# Autodesk Inventor assembly: КВ33.044.900 - Клапан присоски впускной
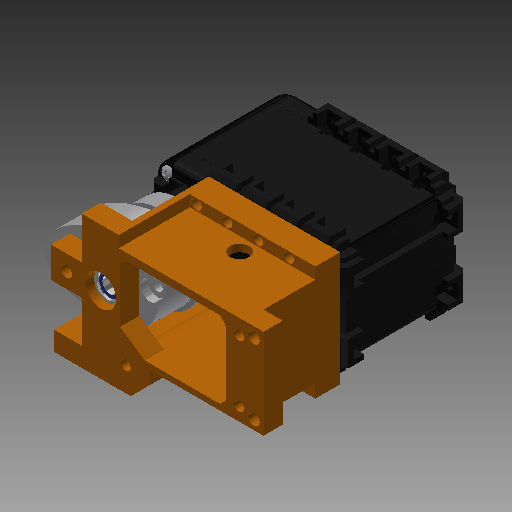
[picture p0: Inventor's stored thumbnail of the model, 512x512]
Saved by Autodesk Inventor 2019 (Build 230136000, 136)
## iProperties
Created: 2019-08-25
Part Number: КВ33.044.900 - Клапан присоски впускной
Material: Типовые
Document SubType Name: Assembly
Designer: Петров Иван
Mass: 93.2423 g
Surface Area: 263.543 cm^2
Volume: 60.5014 cm^3
Density: 1.54116 g/cm^3
Author: Петров Иван
## Documents named in this file (6)
- E:\IVAN\Kvantoriada2019\optimal_gripper\hardware\КВ33.044.900 - Клапан присоски впускной.iam
- E:\IVAN\Kvantoriada2019\optimal_gripper\hardware\КВ33.044.901  - Опора клапана присоски.ipt
- E:\IVAN\Kvantoriada2019\optimal_gripper\hardware\Стандартные изделия\Сервомотор Dynamixel AX-12A\AX-12.iam
- E:\IVAN\Kvantoriada2019\optimal_gripper\hardware\КВ33.044.902 - Кулачок дисковый.ipt
- E:\IVAN\Kvantoriada2019\optimal_gripper\hardware\Стандартные изделия\Подшипник 4x8x3.ipt
- E:\IVAN\Kvantoriada2019\optimal_gripper\hardware\Стандартные изделия\Проставка 4 мм.ipt
## Components (5 placed, 5 different names)
1. КВ33.044.901  - Опора клапана присоски:1 — Заподлицо:1, Совмещение:9, Совмещение:10, Совмещение:11, Совмещение:12
2. AX-12:1 [sub-assembly] — Совмещение:10, Совмещение:11, Совмещение:12, Совмещение:15, Совмещение:16
3. Дисковый кулачок:1 — Совмещение:14, Совмещение:17, Совмещение:18
4. Подшипник 4x8x3:1 — Заподлицо:1, Совмещение:9, Совмещение:14
5. Проставка 4 мм:1 — Совмещение:15, Совмещение:16, Совмещение:17, Совмещение:18
## Relationships (10: Mate 9, Flush 1)
- Заподлицо:1 [Flush]: КВ33.044.901  - Опора клапана присоски:1 ↔ Подшипник 4x8x3:1
- Совмещение:9 [Mate]: КВ33.044.901  - Опора клапана присоски:1 ↔ Подшипник 4x8x3:1
- Совмещение:10 [Mate]: КВ33.044.901  - Опора клапана присоски:1 ↔ AX-12:1
- Совмещение:11 [Mate]: КВ33.044.901  - Опора клапана присоски:1 ↔ AX-12:1
- Совмещение:12 [Mate]: КВ33.044.901  - Опора клапана присоски:1 ↔ AX-12:1
- Совмещение:14 [Mate]: Дисковый кулачок:1 ↔ Подшипник 4x8x3:1
- Совмещение:15 [Mate]: AX-12:1 ↔ Проставка 4 мм:1
- Совмещение:16 [Mate]: AX-12:1 ↔ Проставка 4 мм:1
- Совмещение:17 [Mate]: Дисковый кулачок:1 ↔ Проставка 4 мм:1
- Совмещение:18 [Mate]: Дисковый кулачок:1 ↔ Проставка 4 мм:1
